# Autodesk Inventor assembly: 조립
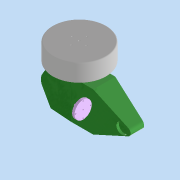
[picture p0: Inventor's stored thumbnail of the model, 180x180]
Saved by Autodesk Inventor 2020 (Build 240168000, 168)
## iProperties
Created: 2020-05-07
Part Number: 조립
Document SubType Name: Assembly
Designer: sbahn
Author: sbahn
## Documents named in this file (10)
- D:\학교 과제\졸업과제\설계\로봇\모델링\조립.iam
- D:\학교 과제\졸업과제\설계\로봇\모델링\본체.ipt
- D:\학교 과제\졸업과제\설계\로봇\모델링\지름 모터 커버.ipt
- D:\학교 과제\졸업과제\설계\로봇\모델링\모터 커버.ipt
- D:\학교 과제\졸업과제\설계\로봇\모델링\전자부품\충방전\충방전.iam
- D:\학교 과제\졸업과제\설계\로봇\모델링\메인 스퍼기어.ipt
- D:\학교 과제\졸업과제\설계\로봇\모델링\메인 스퍼기어 부시.ipt
- D:\학교 과제\졸업과제\설계\로봇\모델링\메인 바퀴 간격링.ipt
- D:\학교 과제\졸업과제\설계\로봇\모델링\메인 바퀴 서포터.ipt
- D:\학교 과제\졸업과제\설계\로봇\모델링\바퀴_MIR.ipt
## Components (9 placed, 9 different names)
1. 본체:1 — 플러쉬:1, 플러쉬:2, 플러쉬:3, 메이트:1, 메이트:2, 메이트:3, 메이트:4, 메이트:5, 메이트:6, 메이트:7, 플러쉬:4, 메이트:8, 메이트:13, 메이트:14
2. 지름 모터 커버:1 — 메이트:1, 메이트:2, 메이트:3
3. 모터 커버:1 — 메이트:4, 메이트:5, 메이트:6
4. 충방전:1 [sub-assembly] — 메이트:7, 플러쉬:4, 메이트:8
5. 메인 스퍼기어:1 — 메이트:9, 메이트:10, 메이트:11, 메이트:12
6. 메인 스퍼기어 부시:1 — 메이트:9, 메이트:10, 메이트:13, 메이트:14
7. 메인 바퀴 간격링:1 — 메이트:11, 메이트:12, 메이트:15, 메이트:16, 메이트:17
8. 메인 바퀴 서포터:1
9. 바퀴_MIR:1 — 메이트:15, 메이트:16, 메이트:17
## Relationships (21: Mate 17, Flush 4)
- 플러쉬:1 [Flush]: 본체:1
- 플러쉬:2 [Flush]: 본체:1
- 플러쉬:3 [Flush]: 본체:1
- 메이트:1 [Mate]: 본체:1 ↔ 지름 모터 커버:1
- 메이트:2 [Mate]: 본체:1 ↔ 지름 모터 커버:1
- 메이트:3 [Mate]: 본체:1 ↔ 지름 모터 커버:1
- 메이트:4 [Mate]: 본체:1 ↔ 모터 커버:1
- 메이트:5 [Mate]: 본체:1 ↔ 모터 커버:1
- 메이트:6 [Mate]: 본체:1 ↔ 모터 커버:1
- 메이트:7 [Mate]: 본체:1 ↔ 충방전:1
- 플러쉬:4 [Flush]: 본체:1 ↔ 충방전:1
- 메이트:8 [Mate]: 본체:1 ↔ 충방전:1
- 메이트:9 [Mate]: 메인 스퍼기어:1 ↔ 메인 스퍼기어 부시:1
- 메이트:10 [Mate]: 메인 스퍼기어:1 ↔ 메인 스퍼기어 부시:1
- 메이트:11 [Mate]: 메인 스퍼기어:1 ↔ 메인 바퀴 간격링:1
- 메이트:12 [Mate]: 메인 스퍼기어:1 ↔ 메인 바퀴 간격링:1
- 메이트:13 [Mate]: 본체:1 ↔ 메인 스퍼기어 부시:1
- 메이트:14 [Mate]: 본체:1 ↔ 메인 스퍼기어 부시:1
- 메이트:15 [Mate]: 메인 바퀴 간격링:1 ↔ 바퀴_MIR:1
- 메이트:16 [Mate]: 메인 바퀴 간격링:1 ↔ 바퀴_MIR:1
- 메이트:17 [Mate]: 메인 바퀴 간격링:1 ↔ 바퀴_MIR:1
